# Autodesk Inventor assembly: Сборка1
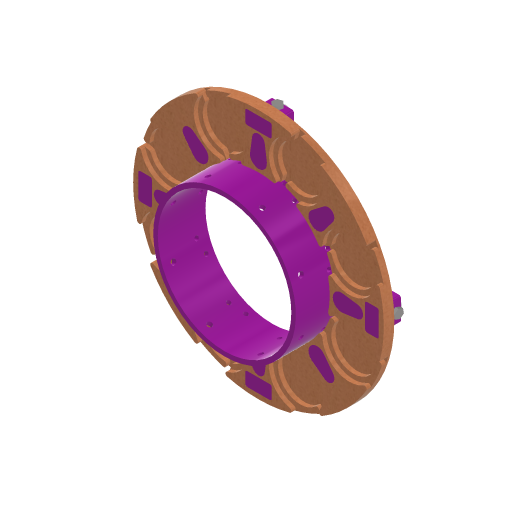
[picture p0: Inventor's stored thumbnail of the model, 512x512]
Saved by Autodesk Inventor 2023 (Build 270158000, 158)
## iProperties
Created: 2023-03-21
Part Number: Сборка1
Document SubType Name: Assembly
Designer: Admin
Author: Admin
## Documents named in this file (9)
- C:\Users\aleks\OneDrive\Рабочий стол\Хроматографический сортировщик\Детали\Хроматографичекий сортировщик.iam
- C:\Users\aleks\OneDrive\Рабочий стол\Хроматографический сортировщик\Детали\Барабан.ipt
- C:\Users\aleks\OneDrive\Рабочий стол\Хроматографический сортировщик\Детали\Короб для подшипника.ipt
- C:\Users\aleks\OneDrive\Рабочий стол\Хроматографический сортировщик\Детали\Покупные\Подшипник.ipt
- C:\Users\aleks\OneDrive\Рабочий стол\Хроматографический сортировщик\Детали\Покупные\Болт М5.ipt
- C:\Users\aleks\OneDrive\Рабочий стол\Хроматографический сортировщик\Детали\Покупные\Гайка М5 стопорная.ipt
- C:\Users\aleks\OneDrive\Рабочий стол\Хроматографический сортировщик\Детали\Покупные\Магнит.ipt
- C:\Users\aleks\OneDrive\Рабочий стол\Хроматографический сортировщик\Детали\Капсуль.ipt
- C:\Users\aleks\OneDrive\Рабочий стол\Хроматографический сортировщик\Детали\Покупные\Болт М5 круглый.ipt
## Components (49 placed, 8 different names)
1. Барабан:1 — Совмещение:9, Совмещение:10, Совмещение:11, Совмещение:12, Совмещение:13, Совмещение:14, Совмещение:15, Совмещение:16, Заподлицо:1, Заподлицо:2, Заподлицо:3, Заподлицо:4, Совмещение:57, Совмещение:58, Заподлицо:13, Совмещение:62, Совмещение:63, Совмещение:68, Совмещение:69, Заподлицо:15, Совмещение:70, Совмещение:71, Совмещение:76, Совмещение:77, Заподлицо:16, Совмещение:78, Совмещение:79, Заподлицо:17, Совмещение:84, Совмещение:85, Совмещение:102, Заподлицо:18, Совмещение:103, Совмещение:104, Заподлицо:19, Совмещение:105, Совмещение:106, Совмещение:107, Заподлицо:20, Совмещение:108, Совмещение:109, Заподлицо:21, Совмещение:111, Совмещение:112, Совмещение:113, Совмещение:114, Совмещение:115, Совмещение:116, Совмещение:117, Совмещение:118, Совмещение:119
2. Короб для подшипника:1 — Совмещение:9, Совмещение:10, Заподлицо:4, Совмещение:17, Совмещение:21, Совмещение:27, Совмещение:32, Совмещение:34, Совмещение:37
3. Короб для подшипника:2 — Совмещение:11, Совмещение:12, Заподлицо:3, Совмещение:19, Совмещение:23, Совмещение:28, Совмещение:29, Совмещение:36, Совмещение:40
4. Короб для подшипника:3 — Совмещение:13, Совмещение:14, Заподлицо:2, Совмещение:20, Совмещение:24, Совмещение:25, Совмещение:30, Совмещение:35, Совмещение:39
5. Короб для подшипника:4 — Совмещение:15, Совмещение:16, Заподлицо:1, Совмещение:18, Совмещение:22, Совмещение:26, Совмещение:31, Совмещение:33, Совмещение:38
6. Подшипник:1 — Совмещение:18, Совмещение:22
7. Подшипник:2 — Совмещение:20, Совмещение:24
8. Подшипник:3 — Совмещение:19, Совмещение:23
9. Подшипник:4 — Совмещение:17, Совмещение:21
10. Болт М5:1 — Совмещение:25, Совмещение:35
11. Гайка М5 стопорная:1 — Совмещение:30, Совмещение:39
12. Болт М5:2 — Совмещение:26, Совмещение:33
13. Гайка М5 стопорная:2 — Совмещение:31, Совмещение:38
14. Болт М5:3 — Совмещение:27, Совмещение:34
15. Гайка М5 стопорная:3 — Совмещение:29, Совмещение:40
16. Болт М5:4 — Совмещение:28, Совмещение:36
17. Гайка М5 стопорная:4 — Совмещение:32, Совмещение:37
18. Магнит:1 — Совмещение:94, Совмещение:95
19. Магнит:2 — Совмещение:66, Совмещение:67
20. Магнит:3 — Совмещение:59, Заподлицо:14
21. Магнит:4 — Совмещение:88, Совмещение:89
22. Магнит:5 — Совмещение:90, Совмещение:91
23. Магнит:6 — Совмещение:82, Совмещение:83
24. Магнит:7 — Совмещение:100, Совмещение:101
25. Магнит:8 — Совмещение:72, Совмещение:73
26. Капсуль:1 — Совмещение:57, Совмещение:58, Заподлицо:13, Совмещение:59, Заподлицо:14, Совмещение:60, Совмещение:61, Угол:1
27. Гайка М5 стопорная:5 — Совмещение:60, Совмещение:61, Угол:1
28. Болт М5 круглый:1 — Совмещение:62, Совмещение:63
29. Капсуль:2 — Совмещение:64, Угол:2, Совмещение:65, Совмещение:66, Совмещение:67, Совмещение:68, Совмещение:69, Заподлицо:15
30. Капсуль:3 — Совмещение:90, Совмещение:91, Совмещение:92, Угол:6, Совмещение:93, Совмещение:108, Совмещение:109, Заподлицо:21
31. Капсуль:4 — Совмещение:72, Совмещение:73, Совмещение:74, Угол:3, Совмещение:75, Совмещение:76, Совмещение:77, Заподлицо:16
32. Капсуль:5 — Совмещение:80, Угол:4, Совмещение:81, Совмещение:82, Совмещение:83, Заподлицо:17, Совмещение:84, Совмещение:85
33. Капсуль:6 — Совмещение:86, Угол:5, Совмещение:87, Совмещение:88, Совмещение:89, Совмещение:102, Заподлицо:18, Совмещение:103
34. Капсуль:7 — Совмещение:94, Совмещение:95, Совмещение:96, Угол:7, Совмещение:97, Совмещение:104, Заподлицо:19, Совмещение:105
35. Капсуль:8 — Совмещение:98, Угол:8, Совмещение:99, Совмещение:100, Совмещение:101, Совмещение:106, Совмещение:107, Заподлицо:20
36. Болт М5 круглый:2 — Совмещение:114, Совмещение:115
37. Гайка М5 стопорная:6 — Совмещение:98, Угол:8, Совмещение:99
38. Болт М5 круглый:3 — Совмещение:112, Совмещение:113
39. Гайка М5 стопорная:7 — Совмещение:96, Угол:7, Совмещение:97
40. Болт М5 круглый:4 — Совмещение:78, Совмещение:79
41. Гайка М5 стопорная:8 — Совмещение:86, Угол:5, Совмещение:87, Совмещение:110
42. Болт М5 круглый:5 — Совмещение:118, Совмещение:119
43. Гайка М5 стопорная:9 — Совмещение:80, Угол:4, Совмещение:81
44. Болт М5 круглый:6 — Совмещение:110, Совмещение:111
45. Гайка М5 стопорная:10 — Совмещение:92, Угол:6, Совмещение:93
46. Болт М5 круглый:7 — Совмещение:116, Совмещение:117
47. Гайка М5 стопорная:11 — Совмещение:74, Угол:3, Совмещение:75
48. Болт М5 круглый:8 — Совмещение:70, Совмещение:71
49. Гайка М5 стопорная:12 — Совмещение:64, Угол:2, Совмещение:65
## Relationships (116: Mate 95, Flush 13, Angle 8)
- Совмещение:9 [Mate]: Барабан:1 ↔ Короб для подшипника:1
- Совмещение:10 [Mate]: Барабан:1 ↔ Короб для подшипника:1
- Совмещение:11 [Mate]: Барабан:1 ↔ Короб для подшипника:2
- Совмещение:12 [Mate]: Барабан:1 ↔ Короб для подшипника:2
- Совмещение:13 [Mate]: Барабан:1 ↔ Короб для подшипника:3
- Совмещение:14 [Mate]: Барабан:1 ↔ Короб для подшипника:3
- Совмещение:15 [Mate]: Барабан:1 ↔ Короб для подшипника:4
- Совмещение:16 [Mate]: Барабан:1 ↔ Короб для подшипника:4
- Заподлицо:1 [Flush]: Барабан:1 ↔ Короб для подшипника:4
- Заподлицо:2 [Flush]: Барабан:1 ↔ Короб для подшипника:3
- Заподлицо:3 [Flush]: Барабан:1 ↔ Короб для подшипника:2
- Заподлицо:4 [Flush]: Барабан:1 ↔ Короб для подшипника:1
- Совмещение:17 [Mate]: Короб для подшипника:1 ↔ Подшипник:4
- Совмещение:18 [Mate]: Короб для подшипника:4 ↔ Подшипник:1
- Совмещение:19 [Mate]: Короб для подшипника:2 ↔ Подшипник:3
- Совмещение:20 [Mate]: Короб для подшипника:3 ↔ Подшипник:2
- Совмещение:21 [Mate] (0.5 mm): Короб для подшипника:1 ↔ Подшипник:4
- Совмещение:22 [Mate] (0.5 mm): Короб для подшипника:4 ↔ Подшипник:1
- Совмещение:23 [Mate] (0.5 mm): Короб для подшипника:2 ↔ Подшипник:3
- Совмещение:24 [Mate] (0.5 mm): Короб для подшипника:3 ↔ Подшипник:2
- Совмещение:25 [Mate]: Короб для подшипника:3 ↔ Болт М5:1
- Совмещение:26 [Mate]: Короб для подшипника:4 ↔ Болт М5:2
- Совмещение:27 [Mate]: Короб для подшипника:1 ↔ Болт М5:3
- Совмещение:28 [Mate]: Короб для подшипника:2 ↔ Болт М5:4
- Совмещение:29 [Mate]: Короб для подшипника:2 ↔ Гайка М5 стопорная:3
- Совмещение:30 [Mate]: Короб для подшипника:3 ↔ Гайка М5 стопорная:1
- Совмещение:31 [Mate]: Короб для подшипника:4 ↔ Гайка М5 стопорная:2
- Совмещение:32 [Mate]: Короб для подшипника:1 ↔ Гайка М5 стопорная:4
- Совмещение:33 [Mate]: Короб для подшипника:4 ↔ Болт М5:2
- Совмещение:34 [Mate]: Короб для подшипника:1 ↔ Болт М5:3
- Совмещение:35 [Mate]: Короб для подшипника:3 ↔ Болт М5:1
- Совмещение:36 [Mate]: Короб для подшипника:2 ↔ Болт М5:4
- Совмещение:37 [Mate]: Короб для подшипника:1 ↔ Гайка М5 стопорная:4
- Совмещение:38 [Mate]: Короб для подшипника:4 ↔ Гайка М5 стопорная:2
- Совмещение:39 [Mate]: Короб для подшипника:3 ↔ Гайка М5 стопорная:1
- Совмещение:40 [Mate]: Короб для подшипника:2 ↔ Гайка М5 стопорная:3
- Совмещение:57 [Mate]: Барабан:1 ↔ Капсуль:1
- Совмещение:58 [Mate]: Барабан:1 ↔ Капсуль:1
- Заподлицо:13 [Flush]: Барабан:1 ↔ Капсуль:1
- Совмещение:59 [Mate]: Магнит:3 ↔ Капсуль:1
- Заподлицо:14 [Flush]: Магнит:3 ↔ Капсуль:1
- Совмещение:60 [Mate]: Капсуль:1 ↔ Гайка М5 стопорная:5
- Совмещение:61 [Mate]: Капсуль:1 ↔ Гайка М5 стопорная:5
- Угол:1 [Angle] (0 deg): Капсуль:1 ↔ Гайка М5 стопорная:5
- Совмещение:62 [Mate]: Барабан:1 ↔ Болт М5 круглый:1
- Совмещение:63 [Mate]: Барабан:1 ↔ Болт М5 круглый:1
- Совмещение:64 [Mate]: Капсуль:2 ↔ Гайка М5 стопорная:12
- Угол:2 [Angle] (0 deg): Капсуль:2 ↔ Гайка М5 стопорная:12
- Совмещение:65 [Mate]: Капсуль:2 ↔ Гайка М5 стопорная:12
- Совмещение:66 [Mate]: Магнит:2 ↔ Капсуль:2
- Совмещение:67 [Mate]: Магнит:2 ↔ Капсуль:2
- Совмещение:68 [Mate]: Барабан:1 ↔ Капсуль:2
- Совмещение:69 [Mate]: Барабан:1 ↔ Капсуль:2
- Заподлицо:15 [Flush]: Барабан:1 ↔ Капсуль:2
- Совмещение:70 [Mate]: Барабан:1 ↔ Болт М5 круглый:8
- Совмещение:71 [Mate]: Барабан:1 ↔ Болт М5 круглый:8
- Совмещение:72 [Mate]: Магнит:8 ↔ Капсуль:4
- Совмещение:73 [Mate]: Магнит:8 ↔ Капсуль:4
- Совмещение:74 [Mate]: Капсуль:4 ↔ Гайка М5 стопорная:11
- Угол:3 [Angle] (0 deg): Капсуль:4 ↔ Гайка М5 стопорная:11
- Совмещение:75 [Mate]: Капсуль:4 ↔ Гайка М5 стопорная:11
- Совмещение:76 [Mate]: Барабан:1 ↔ Капсуль:4
- Совмещение:77 [Mate]: Барабан:1 ↔ Капсуль:4
- Заподлицо:16 [Flush]: Барабан:1 ↔ Капсуль:4
- Совмещение:78 [Mate]: Барабан:1 ↔ Болт М5 круглый:4
- Совмещение:79 [Mate]: Барабан:1 ↔ Болт М5 круглый:4
- Совмещение:80 [Mate]: Капсуль:5 ↔ Гайка М5 стопорная:9
- Угол:4 [Angle] (0 deg): Капсуль:5 ↔ Гайка М5 стопорная:9
- Совмещение:81 [Mate]: Капсуль:5 ↔ Гайка М5 стопорная:9
- Совмещение:82 [Mate]: Магнит:6 ↔ Капсуль:5
- Совмещение:83 [Mate]: Магнит:6 ↔ Капсуль:5
- Заподлицо:17 [Flush]: Барабан:1 ↔ Капсуль:5
- Совмещение:84 [Mate]: Барабан:1 ↔ Капсуль:5
- Совмещение:85 [Mate]: Барабан:1 ↔ Капсуль:5
- Совмещение:86 [Mate]: Капсуль:6 ↔ Гайка М5 стопорная:8
- Угол:5 [Angle] (0 deg): Капсуль:6 ↔ Гайка М5 стопорная:8
- Совмещение:87 [Mate]: Капсуль:6 ↔ Гайка М5 стопорная:8
- Совмещение:88 [Mate]: Магнит:4 ↔ Капсуль:6
- Совмещение:89 [Mate]: Магнит:4 ↔ Капсуль:6
- Совмещение:90 [Mate]: Магнит:5 ↔ Капсуль:3
- Совмещение:91 [Mate]: Магнит:5 ↔ Капсуль:3
- Совмещение:92 [Mate]: Капсуль:3 ↔ Гайка М5 стопорная:10
- Угол:6 [Angle] (0 deg): Капсуль:3 ↔ Гайка М5 стопорная:10
- Совмещение:93 [Mate]: Капсуль:3 ↔ Гайка М5 стопорная:10
- Совмещение:94 [Mate]: Магнит:1 ↔ Капсуль:7
- Совмещение:95 [Mate]: Магнит:1 ↔ Капсуль:7
- Совмещение:96 [Mate]: Капсуль:7 ↔ Гайка М5 стопорная:7
- Угол:7 [Angle] (0 deg): Капсуль:7 ↔ Гайка М5 стопорная:7
- Совмещение:97 [Mate]: Капсуль:7 ↔ Гайка М5 стопорная:7
- Совмещение:98 [Mate]: Капсуль:8 ↔ Гайка М5 стопорная:6
- Угол:8 [Angle] (0 deg): Капсуль:8 ↔ Гайка М5 стопорная:6
- Совмещение:99 [Mate]: Капсуль:8 ↔ Гайка М5 стопорная:6
- Совмещение:100 [Mate]: Магнит:7 ↔ Капсуль:8
- Совмещение:101 [Mate]: Магнит:7 ↔ Капсуль:8
- Совмещение:102 [Mate]: Барабан:1 ↔ Капсуль:6
- Заподлицо:18 [Flush]: Барабан:1 ↔ Капсуль:6
- Совмещение:103 [Mate]: Барабан:1 ↔ Капсуль:6
- Совмещение:104 [Mate]: Барабан:1 ↔ Капсуль:7
- Заподлицо:19 [Flush]: Барабан:1 ↔ Капсуль:7
- Совмещение:105 [Mate]: Барабан:1 ↔ Капсуль:7
- Совмещение:106 [Mate]: Барабан:1 ↔ Капсуль:8
- Совмещение:107 [Mate]: Барабан:1 ↔ Капсуль:8
- Заподлицо:20 [Flush]: Барабан:1 ↔ Капсуль:8
- Совмещение:108 [Mate]: Барабан:1 ↔ Капсуль:3
- Совмещение:109 [Mate]: Барабан:1 ↔ Капсуль:3
- Заподлицо:21 [Flush]: Барабан:1 ↔ Капсуль:3
- Совмещение:110 [Mate]: Гайка М5 стопорная:8 ↔ Болт М5 круглый:6
- Совмещение:111 [Mate]: Барабан:1 ↔ Болт М5 круглый:6
- Совмещение:112 [Mate]: Барабан:1 ↔ Болт М5 круглый:3
- Совмещение:113 [Mate]: Барабан:1 ↔ Болт М5 круглый:3
- Совмещение:114 [Mate]: Барабан:1 ↔ Болт М5 круглый:2
- Совмещение:115 [Mate]: Барабан:1 ↔ Болт М5 круглый:2
- Совмещение:116 [Mate]: Барабан:1 ↔ Болт М5 круглый:7
- Совмещение:117 [Mate]: Барабан:1 ↔ Болт М5 круглый:7
- Совмещение:118 [Mate]: Барабан:1 ↔ Болт М5 круглый:5
- Совмещение:119 [Mate]: Барабан:1 ↔ Болт М5 круглый:5
